# Autodesk Inventor assembly: Wheel Assembly Right
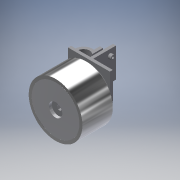
[picture p0: Inventor's stored thumbnail of the model, 180x180]
Saved by Autodesk Inventor 2018 (Build 220112000, 112)
## iProperties
Created: 2017-11-23
Part Number: Wheel Assembly Right
Document SubType Name: Assembly
Designer: prakh
Author: prakh
## Documents named in this file (16)
- D:\GIT\ModernMobility\CADS\Clutch Wheel compact\Wheel Assembly Right.iam
- D:\GIT\ModernMobility\CADS\Clutch Wheel compact\wheel hub.ipt
- D:\GIT\ModernMobility\CADS\Clutch Wheel compact\wheel ring.ipt
- D:\GIT\ModernMobility\CADS\Clutch Wheel compact\clutch plate.ipt
- D:\GIT\ModernMobility\CADS\Clutch Wheel compact\ball bearing ball 0.25in.ipt
- D:\GIT\ModernMobility\CADS\Clutch Wheel compact\mounting plate.ipt
- D:\GIT\ModernMobility\CADS\Clutch Wheel compact\motor mount 2.ipt
- D:\GIT\ModernMobility\CADS\Clutch Wheel compact\POT.ipt
- D:\GIT\ModernMobility\CADS\Clutch Wheel compact\Spur Gears1.iam
- D:\GIT\ModernMobility\CADS\Clutch Wheel compact\spring cap.ipt
- D:\GIT\ModernMobility\CADS\Clutch Wheel compact\3590s-2.ipt
- D:\GIT\ModernMobility\CADS\Clutch Wheel compact\Spur Gear21 pot.ipt
- D:\GIT\ModernMobility\CADS\Clutch Wheel compact\outer ring.ipt
- D:\GIT\ModernMobility\CADS\Clutch Wheel compact\cage.ipt
- D:\GIT\ModernMobility\CADS\Clutch Wheel compact\outer ring end stop.ipt
- D:\GIT\ModernMobility\CADS\Clutch Wheel compact\clutch washer with spring.ipt
## Components (21 placed, 15 different names)
1. mounting plate:1 — Flush:2, Flush:3, Flush:4, Mate:16, Mate:17, Mate:18, Mate:19, Mate:20, Mate:21, Mate:22, Mate:24, Mate:25, Mate:26, Angle:1, Mate:27, Mate:28, Mate:32, Mate:37, Mate:38, Angle:3, Angle:4, Mate:42
2. wheel hub:1 — Mate:1, Flush:1, Mate:8, Mate:9, Mate:10, Mate:11, Mate:12, Mate:13
3. wheel ring:1 — Mate:1, Flush:1, Mate:2, Mate:16
4. clutch plate:1 — Mate:2, Mate:3, Mate:4, Mate:5, Mate:6, Mate:7, Mate:13, Mate:26, Mate:39
5. ball bearing ball 0.25in:1 — Mate:3, Mate:9
6. ball bearing ball 0.25in:2 — Mate:4, Mate:8
7. ball bearing ball 0.25in:3 — Mate:5, Mate:10
8. ball bearing ball 0.25in:4 — Mate:6, Mate:12
9. ball bearing ball 0.25in:5 — Mate:7, Mate:11
10. motor mount 2:1 — Mate:17, Mate:18, Angle:3
11. POT:1 — Mate:19, Mate:20, Mate:23
12. Spur Gears:1 [sub-assembly] — Mate:21, Mate:22, Mate:23, Mate:24, Tangent:1, Rotation:1
13. spring cap:1 — Mate:25, Angle:1, Tangent:1, Mate:40
14. 3590s-2:1 — Mate:27, Mate:28, Mate:29, Mate:30
15. Spur Gear2:1 — Mate:29, Mate:30, Rotation:1
16. outer ring:2 — Mate:32, Mate:34, Flush:5
17. cage:1 — Mate:35, Flush:6
18. cage:2 — Mate:34, Flush:5, Mate:41
19. outer ring end stop:1 — Mate:35, Mate:37, Flush:6, Mate:38
20. clutch washer with spring:1 — Mate:39, Angle:4, Mate:40
21. ball bearing ball 0.25in:6 — Mate:41, Mate:42
## Relationships (48: Mate 37, Flush 6, Angle 3, Tangent 1, RelateRotation 1)
- Mate:1: wheel hub:1 ↔ wheel ring:1
- Flush:1: wheel hub:1 ↔ wheel ring:1
- Mate:2: wheel ring:1 ↔ clutch plate:1
- Mate:3: clutch plate:1 ↔ ball bearing ball 0.25in:1
- Mate:4: clutch plate:1 ↔ ball bearing ball 0.25in:2
- Mate:5: clutch plate:1 ↔ ball bearing ball 0.25in:3
- Mate:6: clutch plate:1 ↔ ball bearing ball 0.25in:4
- Mate:7: clutch plate:1 ↔ ball bearing ball 0.25in:5
- Mate:8 (1.5875 mm): wheel hub:1 ↔ ball bearing ball 0.25in:2
- Mate:9 (1.5875 mm): wheel hub:1 ↔ ball bearing ball 0.25in:1
- Mate:10 (1.5875 mm): wheel hub:1 ↔ ball bearing ball 0.25in:3
- Mate:11 (1.5875 mm): wheel hub:1 ↔ ball bearing ball 0.25in:5
- Mate:12 (1.5875 mm): wheel hub:1 ↔ ball bearing ball 0.25in:4
- Mate:13 (1.5875 mm): wheel hub:1 ↔ clutch plate:1
- Flush:2: mounting plate:1
- Flush:3: mounting plate:1
- Flush:4: mounting plate:1
- Mate:16: mounting plate:1 ↔ wheel ring:1
- Mate:17: mounting plate:1 ↔ motor mount 2:1
- Mate:18: mounting plate:1 ↔ motor mount 2:1
- Mate:19: mounting plate:1 ↔ POT:1
- Mate:20: mounting plate:1 ↔ POT:1
- Mate:21: mounting plate:1 ↔ Spur Gears:1
- Mate:22: mounting plate:1 ↔ Spur Gears:1
- Mate:23: POT:1 ↔ Spur Gears:1
- Mate:24: mounting plate:1 ↔ Spur Gears:1
- Mate:25: mounting plate:1 ↔ spring cap:1
- Mate:26 (3.175 mm): mounting plate:1 ↔ clutch plate:1
- Angle:1 (0 deg): mounting plate:1 ↔ spring cap:1
- Tangent:1: Spur Gears:1 ↔ spring cap:1
- Mate:27: mounting plate:1 ↔ 3590s-2:1
- Mate:28: mounting plate:1 ↔ 3590s-2:1
- Mate:29: 3590s-2:1 ↔ Spur Gear2:1
- Mate:30: 3590s-2:1 ↔ Spur Gear2:1
- Rotation:1 [RelateRotation] (0.199 ul): Spur Gears:1 ↔ Spur Gear2:1
- Mate:32: mounting plate:1 ↔ outer ring:2
- Mate:34: outer ring:2 ↔ cage:2
- Flush:5: outer ring:2 ↔ cage:2
- Mate:35: cage:1 ↔ outer ring end stop:1
- Mate:37: mounting plate:1 ↔ outer ring end stop:1
- Flush:6: cage:1 ↔ outer ring end stop:1
- Mate:38 (3.175 mm): mounting plate:1 ↔ outer ring end stop:1
- Angle:3 (0 deg): mounting plate:1 ↔ motor mount 2:1
- Mate:39: clutch plate:1 ↔ clutch washer with spring:1
- Angle:4 (0 deg): mounting plate:1 ↔ clutch washer with spring:1
- Mate:40: spring cap:1 ↔ clutch washer with spring:1
- Mate:41: cage:2 ↔ ball bearing ball 0.25in:6
- Mate:42: mounting plate:1 ↔ ball bearing ball 0.25in:6
